# Autodesk Inventor assembly: IMU
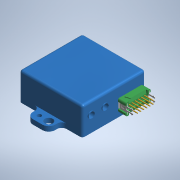
[picture p0: Inventor's stored thumbnail of the model, 180x180]
Saved by Autodesk Inventor 2022.1 (Build 261234000, 234)
## iProperties
Part Number: IMU
Document SubType Name: Ensamblaje
Designer: seb_0
Author: seb_0
## Documents named in this file (3)
- C:\Users\seb_0\Desktop\PDM\ProyectoRobotPallet\IMU\IMU.iam
- C:\Users\seb_0\Desktop\PDM\ProyectoRobotPallet\IMU\Sensor inercial.ipt
- C:\Users\seb_0\Desktop\PDM\ProyectoRobotPallet\IMU\g125-mv11205l1_asm.iam
## Components (2 placed, 2 different names)
1. Sensor inercial:1 — Coincidencia:2, Nivelación:1, Coincidencia:3, Coincidencia:4, Nivelación:2
2. g125-mv11205l1_asm:1 [sub-assembly] — Coincidencia:2, Nivelación:1, Nivelación:2
## Relationships (5: Mate 3, Flush 2)
- Coincidencia:2 [Mate] (-6.6421 mm): Sensor inercial:1 ↔ g125-mv11205l1_asm:1
- Nivelación:1 [Flush] (-1.016 mm): Sensor inercial:1 ↔ g125-mv11205l1_asm:1
- Coincidencia:3 [Mate]: Sensor inercial:1
- Coincidencia:4 [Mate]: Sensor inercial:1
- Nivelación:2 [Flush] (3.1496 mm): Sensor inercial:1 ↔ g125-mv11205l1_asm:1
